# Autodesk Inventor assembly: The Bump
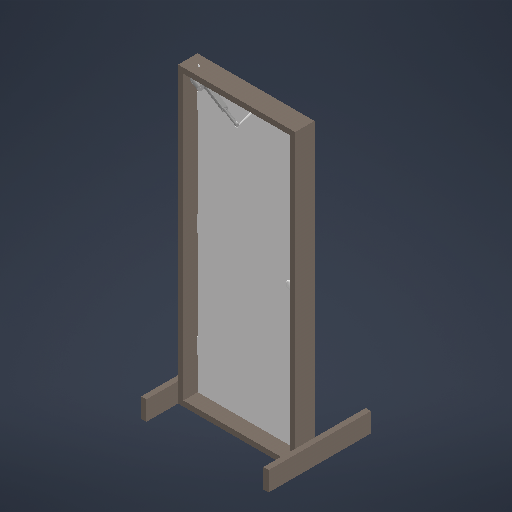
[picture p0: Inventor's stored thumbnail of the model, 512x512]
Saved by Autodesk Inventor 2026.2 (Build 302298010, 298A)
## iProperties
Created: 2026-03-06
Part Number: The Bump
Document SubType Name: Assembly
Designer: brand
Author: brand
## Documents named in this file (24)
- C:\Users\brand\MMAE432\TheBump\The Bump.iam
- C:\Users\brand\MMAE432\TheBump\1518A15_Single Door\1518A15_Single Door\1518A15_Single Door.ipt
- C:\Users\brand\MMAE432\TheBump\DoorFrame.ipt
- C:\Users\brand\MMAE432\TheBump\1494A43_Mortise-Mount Entry Door Template Hinge\1494A43_Mortise-Mount Entry Door Template Hinge\1494A43_Mortise-Mount Entry Door Template Hinge.ipt
- C:\Users\brand\MMAE432\TheBump\DoorFrameBase.ipt
- C:\Users\brand\MMAE432\TheBump\12895A21_Door Knob\12895A21_Door Knob\12895A21_Door Knob.ipt
- C:\Users\brand\MMAE432\TheBump\FA-35(150)(200)-12-9-P\FA-35(150)(200)-12-9-P\FA-35(150)(200)-12-9-P.ipt
- C:\Users\brand\MMAE432\TheBump\LinkageAlign.ipt
- C:\Users\brand\MMAE432\TheBump\91166A250_Zinc-Plated Steel General Purpose Washer\91166A250_Zinc-Plated Steel General Purpose Washer\91166A250_Zinc-Plated Steel General Purpose Washer.ipt
- C:\Users\brand\MMAE432\TheBump\90576A115_Medium-Strength Steel Nylon-Insert Locknut\90576A115_Medium-Strength Steel Nylon-Insert Locknut\90576A115_Medium-Strength Steel Nylon-Insert Locknut.ipt
- C:\Users\brand\MMAE432\TheBump\3799K601_Right-Hand Partially Threaded Rod End Bolt\3799K601_Right-Hand Partially Threaded Rod End Bolt\3799K601_Right-Hand Partially Threaded Rod End Bolt.ipt
- C:\Users\brand\MMAE432\TheBump\7416N19_Internally Threaded Connecting Rod\7416N19_Internally Threaded Connecting Rod\7416N19_Internally Threaded Connecting Rod.ipt
- C:\Users\brand\MMAE432\TheBump\5621N12_Rod End Nut\5621N12_Rod End Nut\5621N12_Rod End Nut.ipt
- C:\Users\brand\MMAE432\TheBump\FA-35(150)(200)-12-9-P\FA-35(150)(200)-12-9-P\FA-35(150)(200)-12-9-P - Cylinder.ipt
- C:\Users\brand\MMAE432\TheBump\DoorFrame2.ipt
- C:\Users\brand\MMAE432\TheBump\1518A15_Single Door\1518A15_Single Door\1518A15_Single Door2.ipt
- C:\Users\brand\MMAE432\TheBump\MB1-P\MB1-P\MB1-P.ipt
- C:\Users\brand\MMAE432\TheBump\91290A209_Black-Oxide Alloy Steel Socket Head Screw\91290A209_Black-Oxide Alloy Steel Socket Head Screw\91290A209_Black-Oxide Alloy Steel Socket Head Screw.ipt
- C:\Users\brand\MMAE432\TheBump\90576A118_Medium-Strength Steel Nylon-Insert Locknut\90576A118_Medium-Strength Steel Nylon-Insert Locknut\90576A118_Medium-Strength Steel Nylon-Insert Locknut.ipt
- C:\Users\brand\MMAE432\TheBump\91280A302_Medium-Strength Class 8.8 Steel Hex Head Screw\91280A302_Medium-Strength Class 8.8 Steel Hex Head Screw\91280A302_Medium-Strength Class 8.8 Steel Hex Head Screw.ipt
- C:\Users\brand\MMAE432\TheBump\BracketSpacer.ipt
- C:\Users\brand\MMAE432\TheBump\ActuatorSpacer.ipt
- C:\Users\brand\MMAE432\TheBump\FA-XXX-S-12-3\FA-XXX-S-12-3\FA-XXX-S-12-3.ipt
- C:\Users\brand\OneDrive\Documents\ActuatorMount.ipt
## Components (72 placed, 23 different names)
1. LinkageAlign:1 — Flush:14
2. 1518A15_Single Door2:2 — Mate:37
3. DoorFrame2:2 — Mate:36, Angle:5
4. DoorFrameBase:5
5. DoorFrameBase:6
6. 12895A21_Door Knob:3
7. 1494A43_Mortise-Mount Entry Door Template Hinge:18
8. 1494A43_Mortise-Mount Entry Door Template Hinge:19
9. 1494A43_Mortise-Mount Entry Door Template Hinge:20
10. 1494A43_Mortise-Mount Entry Door Template Hinge:21
11. 1494A43_Mortise-Mount Entry Door Template Hinge:22
12. 1494A43_Mortise-Mount Entry Door Template Hinge:23
13. FA-XXX-S-12-3:1 — Flush:40, Insert:40, Angle:5
14. ActuatorMount:1 — Flush:40, Mate:36, Mate:37, Insert:40
15. 1518A15_Single Door:1 — Mate:2, Mate:3, Mate:4, Flush:10, Mate:5, Flush:13, Insert:9, Insert:10, Angle:2
16. DoorFrame:1 — Flush:4, Flush:5, Mate:1, Flush:8, Mate:6, Flush:12, Flush:14, Insert:1, Insert:2, Flush:25, Flush:26
17. DoorFrameBase:1 — Flush:4, Flush:5, Flush:7, Flush:9
18. DoorFrameBase:2 — Flush:7, Mate:1, Flush:8, Flush:9
19. 12895A21_Door Knob:1 — Mate:2, Mate:3, Mate:4
20. FA-35(150)(200)-12-9-P:1 — Insert:7, Cylindrical:2
21. 91166A250_Zinc-Plated Steel General Purpose Washer:1 — Insert:2, Insert:4
22. 91166A250_Zinc-Plated Steel General Purpose Washer:2 — Insert:1, Insert:3
23. 90576A115_Medium-Strength Steel Nylon-Insert Locknut:1 — Insert:3
24. 90576A115_Medium-Strength Steel Nylon-Insert Locknut:2 — Insert:6, Insert:7
25. 91166A250_Zinc-Plated Steel General Purpose Washer:3 — Insert:4, Insert:5
26. 91166A250_Zinc-Plated Steel General Purpose Washer:4 — Insert:5, Insert:6
27. 3799K601_Right-Hand Partially Threaded Rod End Bolt:1 — Mate:7, Insert:8, Mate:9, Mate:12, Mate:13
28. 3799K601_Right-Hand Partially Threaded Rod End Bolt:2 — Mate:10, Mate:11
29. 91166A250_Zinc-Plated Steel General Purpose Washer:5 — Insert:8, Tangent:1
30. 90576A115_Medium-Strength Steel Nylon-Insert Locknut:3 — Mate:8, Tangent:2
31. 7416N19_Internally Threaded Connecting Rod:1 — Mate:9, Mate:10, Mate:13, Insert:11, Insert:12
32. 5621N12_Rod End Nut:1 — Insert:10, Angle:1, Angle:2, Mate:11, Insert:13
33. 5621N12_Rod End Nut:2 — Insert:9, Angle:1, Mate:12
34. 90576A115_Medium-Strength Steel Nylon-Insert Locknut:4 — Insert:11
35. 90576A115_Medium-Strength Steel Nylon-Insert Locknut:5 — Insert:12
36. 91166A250_Zinc-Plated Steel General Purpose Washer:6 — Insert:13, Insert:14
37. 90576A115_Medium-Strength Steel Nylon-Insert Locknut:6 — Insert:14
38. FA-35(150)(200)-12-9-P - Cylinder:1 — Mate:8, Tangent:2, Tangent:1, Mate:7, Cylindrical:2
39. 1518A15_Single Door2:1 — Angle:4, Insert:23, Insert:24, Insert:28, Insert:29, Flush:27, Insert:31, Flush:30
40. DoorFrame2:1 — Flush:25, Flush:26, Mate:27, Angle:3, Flush:29
41. DoorFrameBase:3
42. DoorFrameBase:4
43. 12895A21_Door Knob:2
44. FA-35(150)(200)-12-9-P:2 — Insert:21, Insert:25
45. 91166A250_Zinc-Plated Steel General Purpose Washer:7 — Insert:30
46. 91166A250_Zinc-Plated Steel General Purpose Washer:8
47. 90576A115_Medium-Strength Steel Nylon-Insert Locknut:7
48. 90576A115_Medium-Strength Steel Nylon-Insert Locknut:8 — Insert:20, Insert:21
49. 91166A250_Zinc-Plated Steel General Purpose Washer:9
50. 91166A250_Zinc-Plated Steel General Purpose Washer:10 — Insert:22
51. FA-35(150)(200)-12-9-P - Cylinder:2 — Mate:28, Tangent:3
52. MB1-P:1 — Angle:3, Mate:28, Angle:4, Tangent:3, Insert:23, Insert:24, Insert:26, Insert:27
53. 91166A250_Zinc-Plated Steel General Purpose Washer:11 — Insert:20, Insert:22
54. 91290A209_Black-Oxide Alloy Steel Socket Head Screw:1 — Insert:25
55. 90576A118_Medium-Strength Steel Nylon-Insert Locknut:1 — Insert:27
56. 90576A118_Medium-Strength Steel Nylon-Insert Locknut:2 — Insert:26
57. 91280A302_Medium-Strength Class 8.8 Steel Hex Head Screw:1 — Insert:28
58. 91280A302_Medium-Strength Class 8.8 Steel Hex Head Screw:2 — Insert:29
59. BracketSpacer:1 — Flush:27, Insert:31, Flush:30
60. ActuatorSpacer:1 — Flush:29, Insert:30
61. 1494A43_Mortise-Mount Entry Door Template Hinge:6 — Flush:10, Mate:5, Flush:11, Flush:13, Cylindrical:1
62. 1494A43_Mortise-Mount Entry Door Template Hinge:7 — Mate:6, Flush:11, Flush:12, Cylindrical:1
63. 1494A43_Mortise-Mount Entry Door Template Hinge:8
64. 1494A43_Mortise-Mount Entry Door Template Hinge:9
65. 1494A43_Mortise-Mount Entry Door Template Hinge:10
66. 1494A43_Mortise-Mount Entry Door Template Hinge:11
67. 1494A43_Mortise-Mount Entry Door Template Hinge:12
68. 1494A43_Mortise-Mount Entry Door Template Hinge:13 — Mate:27
69. 1494A43_Mortise-Mount Entry Door Template Hinge:14
70. 1494A43_Mortise-Mount Entry Door Template Hinge:15
71. 1494A43_Mortise-Mount Entry Door Template Hinge:16
72. 1494A43_Mortise-Mount Entry Door Template Hinge:17
## Component patterns: (3 elements, first: 1494A43_Mortise-Mount Entry Door Template Hinge:6 + 1494A43_Mortise-Mount Entry Door Template Hinge:7), (3 elements, first: 1494A43_Mortise-Mount Entry Door Template Hinge:12 + 1494A43_Mortise-Mount Entry Door Template Hinge:13)
## Relationships (109: Flush 34, Insert 32, Mate 30, CylindricalJoint 5, Angle 5, Tangent 3)
- Flush:4: DoorFrame:1 ↔ DoorFrameBase:1
- Flush:5: DoorFrame:1 ↔ DoorFrameBase:1
- Flush:7: DoorFrameBase:1 ↔ DoorFrameBase:2
- Mate:1: DoorFrame:1 ↔ DoorFrameBase:2
- Flush:8: DoorFrame:1 ↔ DoorFrameBase:2
- Flush:9: DoorFrameBase:1 ↔ DoorFrameBase:2
- Mate:2: 1518A15_Single Door:1 ↔ 12895A21_Door Knob:1
- Mate:3: 1518A15_Single Door:1 ↔ 12895A21_Door Knob:1
- Mate:4 (15.7226 mm): 1518A15_Single Door:1 ↔ 12895A21_Door Knob:1
- Flush:10 (152.4 mm): 1518A15_Single Door:1 ↔ 1494A43_Mortise-Mount Entry Door Template Hinge:6
- Mate:5: 1518A15_Single Door:1 ↔ 1494A43_Mortise-Mount Entry Door Template Hinge:6
- Mate:6: DoorFrame:1 ↔ 1494A43_Mortise-Mount Entry Door Template Hinge:7
- Flush:11: 1494A43_Mortise-Mount Entry Door Template Hinge:6 ↔ 1494A43_Mortise-Mount Entry Door Template Hinge:7
- Flush:12: DoorFrame:1 ↔ 1494A43_Mortise-Mount Entry Door Template Hinge:7
- Flush:13: 1518A15_Single Door:1 ↔ 1494A43_Mortise-Mount Entry Door Template Hinge:6
- Cylindrical:1: 1494A43_Mortise-Mount Entry Door Template Hinge:6 ↔ 1494A43_Mortise-Mount Entry Door Template Hinge:7
- Flush:14: LinkageAlign:1 ↔ DoorFrame:1
- Insert:1: DoorFrame:1 ↔ 91166A250_Zinc-Plated Steel General Purpose Washer:2
- Insert:2: DoorFrame:1 ↔ 91166A250_Zinc-Plated Steel General Purpose Washer:1
- Insert:3: 91166A250_Zinc-Plated Steel General Purpose Washer:2 ↔ 90576A115_Medium-Strength Steel Nylon-Insert Locknut:1
- Insert:4: 91166A250_Zinc-Plated Steel General Purpose Washer:1 ↔ 91166A250_Zinc-Plated Steel General Purpose Washer:3
- Insert:5: 91166A250_Zinc-Plated Steel General Purpose Washer:3 ↔ 91166A250_Zinc-Plated Steel General Purpose Washer:4
- Insert:6: 90576A115_Medium-Strength Steel Nylon-Insert Locknut:2 ↔ 91166A250_Zinc-Plated Steel General Purpose Washer:4
- Insert:7: FA-35(150)(200)-12-9-P:1 ↔ 90576A115_Medium-Strength Steel Nylon-Insert Locknut:2
- Mate:7: 3799K601_Right-Hand Partially Threaded Rod End Bolt:1 ↔ FA-35(150)(200)-12-9-P - Cylinder:1
- Insert:8: 3799K601_Right-Hand Partially Threaded Rod End Bolt:1 ↔ 91166A250_Zinc-Plated Steel General Purpose Washer:5
- Tangent:1: 91166A250_Zinc-Plated Steel General Purpose Washer:5 ↔ FA-35(150)(200)-12-9-P - Cylinder:1
- Mate:8: 90576A115_Medium-Strength Steel Nylon-Insert Locknut:3 ↔ FA-35(150)(200)-12-9-P - Cylinder:1
- Tangent:2: 90576A115_Medium-Strength Steel Nylon-Insert Locknut:3 ↔ FA-35(150)(200)-12-9-P - Cylinder:1
- Mate:9: 3799K601_Right-Hand Partially Threaded Rod End Bolt:1 ↔ 7416N19_Internally Threaded Connecting Rod:1
- Mate:10: 3799K601_Right-Hand Partially Threaded Rod End Bolt:2 ↔ 7416N19_Internally Threaded Connecting Rod:1
- Insert:9: 1518A15_Single Door:1 ↔ 5621N12_Rod End Nut:2
- Insert:10: 1518A15_Single Door:1 ↔ 5621N12_Rod End Nut:1
- Angle:1 (0 deg): 5621N12_Rod End Nut:1 ↔ 5621N12_Rod End Nut:2
- Angle:2 (0 deg): 1518A15_Single Door:1 ↔ 5621N12_Rod End Nut:1
- Mate:11: 3799K601_Right-Hand Partially Threaded Rod End Bolt:2 ↔ 5621N12_Rod End Nut:1
- Mate:12 (187.5536 mm): 3799K601_Right-Hand Partially Threaded Rod End Bolt:1 ↔ 5621N12_Rod End Nut:2
- Mate:13 (4.572 mm): 3799K601_Right-Hand Partially Threaded Rod End Bolt:1 ↔ 7416N19_Internally Threaded Connecting Rod:1
- Insert:11: 7416N19_Internally Threaded Connecting Rod:1 ↔ 90576A115_Medium-Strength Steel Nylon-Insert Locknut:4
- Insert:12: 7416N19_Internally Threaded Connecting Rod:1 ↔ 90576A115_Medium-Strength Steel Nylon-Insert Locknut:5
- Insert:13: 5621N12_Rod End Nut:1 ↔ 91166A250_Zinc-Plated Steel General Purpose Washer:6
- Insert:14: 91166A250_Zinc-Plated Steel General Purpose Washer:6 ↔ 90576A115_Medium-Strength Steel Nylon-Insert Locknut:6
- Cylindrical:2: FA-35(150)(200)-12-9-P:1 ↔ FA-35(150)(200)-12-9-P - Cylinder:1
- [Flush]: DoorFrame2:1 ↔ DoorFrameBase:3
- [Flush]: DoorFrame2:1 ↔ DoorFrameBase:3
- [Flush]: DoorFrameBase:3 ↔ DoorFrameBase:4
- [Mate]: DoorFrame2:1 ↔ DoorFrameBase:4
- [Flush]: DoorFrame2:1 ↔ DoorFrameBase:4
- [Flush]: DoorFrameBase:3 ↔ DoorFrameBase:4
- [Mate]: 1518A15_Single Door2:1 ↔ 12895A21_Door Knob:2
- [Mate]: 1518A15_Single Door2:1 ↔ 12895A21_Door Knob:2
- [Mate] (15.7226 mm): 1518A15_Single Door2:1 ↔ 12895A21_Door Knob:2
- [Flush] (152.4 mm): 1518A15_Single Door2:1 ↔ 1494A43_Mortise-Mount Entry Door Template Hinge:12
- [Mate]: 1518A15_Single Door2:1 ↔ 1494A43_Mortise-Mount Entry Door Template Hinge:12
- [Mate]: DoorFrame2:1 ↔ 1494A43_Mortise-Mount Entry Door Template Hinge:13
- [Flush]: 1494A43_Mortise-Mount Entry Door Template Hinge:12 ↔ 1494A43_Mortise-Mount Entry Door Template Hinge:13
- [Flush]: DoorFrame2:1 ↔ 1494A43_Mortise-Mount Entry Door Template Hinge:13
- [Flush]: 1518A15_Single Door2:1 ↔ 1494A43_Mortise-Mount Entry Door Template Hinge:12
- [CylindricalJoint]: 1494A43_Mortise-Mount Entry Door Template Hinge:12 ↔ 1494A43_Mortise-Mount Entry Door Template Hinge:13
- [Insert]: DoorFrame2:1 ↔ 91166A250_Zinc-Plated Steel General Purpose Washer:8
- [Insert]: DoorFrame2:1 ↔ 91166A250_Zinc-Plated Steel General Purpose Washer:7
- [Insert]: 91166A250_Zinc-Plated Steel General Purpose Washer:8 ↔ 90576A115_Medium-Strength Steel Nylon-Insert Locknut:7
- [Insert]: 91166A250_Zinc-Plated Steel General Purpose Washer:7 ↔ 91166A250_Zinc-Plated Steel General Purpose Washer:9
- [Insert]: 91166A250_Zinc-Plated Steel General Purpose Washer:9 ↔ 91166A250_Zinc-Plated Steel General Purpose Washer:10
- Insert:20: 90576A115_Medium-Strength Steel Nylon-Insert Locknut:8 ↔ 91166A250_Zinc-Plated Steel General Purpose Washer:11
- Insert:21: FA-35(150)(200)-12-9-P:2 ↔ 90576A115_Medium-Strength Steel Nylon-Insert Locknut:8
- [CylindricalJoint]: FA-35(150)(200)-12-9-P:2 ↔ FA-35(150)(200)-12-9-P - Cylinder:2
- Flush:25: DoorFrame:1 ↔ DoorFrame2:1
- Flush:26: DoorFrame:1 ↔ DoorFrame2:1
- Mate:27 (160.528 mm): DoorFrame2:1 ↔ 1494A43_Mortise-Mount Entry Door Template Hinge:13
- Angle:3 (180 deg): DoorFrame2:1 ↔ MB1-P:1
- Mate:28: FA-35(150)(200)-12-9-P - Cylinder:2 ↔ MB1-P:1
- Insert:22: 91166A250_Zinc-Plated Steel General Purpose Washer:10 ↔ 91166A250_Zinc-Plated Steel General Purpose Washer:11
- Angle:4 (180 deg): 1518A15_Single Door2:1 ↔ MB1-P:1
- Tangent:3: FA-35(150)(200)-12-9-P - Cylinder:2 ↔ MB1-P:1
- Insert:23 (49.5554 mm): 1518A15_Single Door2:1 ↔ MB1-P:1
- Insert:24 (49.5554 mm): 1518A15_Single Door2:1 ↔ MB1-P:1
- Insert:25: FA-35(150)(200)-12-9-P:2 ↔ 91290A209_Black-Oxide Alloy Steel Socket Head Screw:1
- Insert:26: MB1-P:1 ↔ 90576A118_Medium-Strength Steel Nylon-Insert Locknut:2
- Insert:27: MB1-P:1 ↔ 90576A118_Medium-Strength Steel Nylon-Insert Locknut:1
- Insert:28: 1518A15_Single Door2:1 ↔ 91280A302_Medium-Strength Class 8.8 Steel Hex Head Screw:1
- Insert:29: 1518A15_Single Door2:1 ↔ 91280A302_Medium-Strength Class 8.8 Steel Hex Head Screw:2
- Flush:27: 1518A15_Single Door2:1 ↔ BracketSpacer:1
- Flush:29: DoorFrame2:1 ↔ ActuatorSpacer:1
- Insert:30: 91166A250_Zinc-Plated Steel General Purpose Washer:7 ↔ ActuatorSpacer:1
- Insert:31: 1518A15_Single Door2:1 ↔ BracketSpacer:1
- Flush:30: 1518A15_Single Door2:1 ↔ BracketSpacer:1
- [Flush]: DoorFrame2:2 ↔ DoorFrameBase:5
- [Flush]: DoorFrame2:2 ↔ DoorFrameBase:5
- [Flush]: DoorFrameBase:5 ↔ DoorFrameBase:6
- [Mate]: DoorFrame2:2 ↔ DoorFrameBase:6
- [Flush]: DoorFrame2:2 ↔ DoorFrameBase:6
- [Flush]: DoorFrameBase:5 ↔ DoorFrameBase:6
- [Mate]: 1518A15_Single Door2:2 ↔ 12895A21_Door Knob:3
- [Mate]: 1518A15_Single Door2:2 ↔ 12895A21_Door Knob:3
- [Mate] (15.7226 mm): 1518A15_Single Door2:2 ↔ 12895A21_Door Knob:3
- [Flush] (152.4 mm): 1518A15_Single Door2:2 ↔ 1494A43_Mortise-Mount Entry Door Template Hinge:18
- [Mate]: 1518A15_Single Door2:2 ↔ 1494A43_Mortise-Mount Entry Door Template Hinge:18
- [Mate]: DoorFrame2:2 ↔ 1494A43_Mortise-Mount Entry Door Template Hinge:19
- [Flush]: 1494A43_Mortise-Mount Entry Door Template Hinge:18 ↔ 1494A43_Mortise-Mount Entry Door Template Hinge:19
- [Flush]: DoorFrame2:2 ↔ 1494A43_Mortise-Mount Entry Door Template Hinge:19
- [Flush]: 1518A15_Single Door2:2 ↔ 1494A43_Mortise-Mount Entry Door Template Hinge:18
- [CylindricalJoint]: 1494A43_Mortise-Mount Entry Door Template Hinge:18 ↔ 1494A43_Mortise-Mount Entry Door Template Hinge:19
- [Mate] (160.528 mm): DoorFrame2:2 ↔ 1494A43_Mortise-Mount Entry Door Template Hinge:19
- Flush:40: FA-XXX-S-12-3:1 ↔ ActuatorMount:1
- Mate:36: DoorFrame2:2 ↔ ActuatorMount:1
- Mate:37 (12.7 mm): 1518A15_Single Door2:2 ↔ ActuatorMount:1
- Insert:40: FA-XXX-S-12-3:1 ↔ ActuatorMount:1
- Angle:5 (180 deg): DoorFrame2:2 ↔ FA-XXX-S-12-3:1
## Named parameters: d101_d12 = 0 mm, d102_d13 = 0 mm, d103_d14 = 0 mm, d104_d15 = 0 mm, d105_d16 = 0 mm, d106_d17 = 15.7226 mm, d107_d7 = 0 mm, d108_d8 = 0 mm, d109_d11 = 0 mm, d110_d97 = -165.968653 deg, d111_d98 = -0.00629 mm, d112_d99 = 228.6 mm, d113_d100 = 0 mm, d114_d92 = -97.92 deg, d115_d93 = 0 deg, d116_d62 = 0 mm, d117_d63 = 0 mm, d118_d64 = 0 mm, d119_d65 = 0 mm, d120_d66 = 0 mm, d121_d68 = 0 mm, d122_d69 = 0 mm, d132_d24 = 152.4 mm, d133_d25 = 0 mm, d134_d26 = 0 mm, d135_d27 = 0 mm, d136_d28 = 0 mm, d137_d29 = 0 mm, d138_d30 = 0 deg, d139_d31 = 0 mm, d209_d103_d14 = 0 mm, d210_d104_d15 = 0 mm, d211_d105_d16 = 0 mm, d212_d106_d17 = 15.7226 mm, d213_d107_d7 = 0 mm, d214_d108_d8 = 0 mm, d215_d109_d11 = 0 mm, d220_d114_d92 = -97.92 deg, d221_d115_d93 = 0 deg, d229_d132_d24 = 152.4 mm, d230_d133_d25 = 0 mm, d231_d134_d26 = 0 mm, d232_d135_d27 = 0 mm, d233_d136_d28 = 0 mm, d234_d137_d29 = 0 mm, d235_d138_d30 = 0 deg, d236_d139_d31 = 0 mm, d237_d155 = 160.528 mm, d238_d101_d12 = 0 mm, d239_d102_d13 = 0 mm
